# Autodesk Inventor assembly: Assembly_Rymapt_Ethoscope
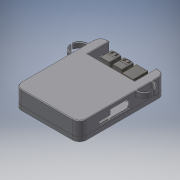
[picture p0: Inventor's stored thumbnail of the model, 180x180]
Saved by Autodesk Inventor 2017 (Build 210142000, 142)
## iProperties
Created: 2017-05-29
Part Number: Assembly_Rymapt_Ethoscope
Document SubType Name: Assembly
Designer: Paolo
Author: Paolo
## Documents named in this file (6)
- E:\Rymapt_projects\Ethoscope\ethoscope_hardware\core_Rymapt\Assembly_Rymapt_Ethoscope.iam
- E:\Rymapt_projects\Ethoscope\ethoscope_hardware\core_Rymapt\LightBox\core_lightBox_new.ipt
- E:\Rymapt_projects\Ethoscope\ethoscope_hardware\arenas\arena_10x1_longTubes\arena_10x1_longTubes.ipt
- E:\Rymapt_projects\Ethoscope\ethoscope_hardware\core_Rymapt\PiCase\lowerPiCase_new.ipt
- E:\Rymapt_projects\Ethoscope\ethoscope_hardware\core\RPi3\RPi3_ModelB.ipt
- E:\Rymapt_projects\Ethoscope\ethoscope_hardware\core_Rymapt\PiCase\upperPiCase_R.ipt
## Components (5 placed, 5 different names)
1. core_lightBox_new:1 — Mate:1, Mate:2, Mate:3, Flush:1, Flush:2
2. arena_10x1_longTubes:1 — Mate:1, Mate:2, Mate:3
3. lowerPiCase_new:1 — Flush:1, Flush:2, Mate:4, Angle:1, Mate:5, Flush:3, Flush:4
4. RPi3_ModelB:1 — Mate:4, Angle:1, Mate:5
5. upperPiCase_R:1 — Flush:3, Flush:4
## Relationships (10: Mate 5, Flush 4, Angle 1)
- Mate:1: core_lightBox_new:1 ↔ arena_10x1_longTubes:1
- Mate:2: core_lightBox_new:1 ↔ arena_10x1_longTubes:1
- Mate:3: core_lightBox_new:1 ↔ arena_10x1_longTubes:1
- Flush:1: core_lightBox_new:1 ↔ lowerPiCase_new:1
- Flush:2: core_lightBox_new:1 ↔ lowerPiCase_new:1
- Mate:4: lowerPiCase_new:1 ↔ RPi3_ModelB:1
- Angle:1 (0 deg): lowerPiCase_new:1 ↔ RPi3_ModelB:1
- Mate:5 (0.2 mm): lowerPiCase_new:1 ↔ RPi3_ModelB:1
- Flush:3: lowerPiCase_new:1 ↔ upperPiCase_R:1
- Flush:4: lowerPiCase_new:1 ↔ upperPiCase_R:1
